# Autodesk Inventor assembly: Assembly1
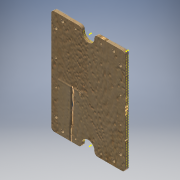
[picture p0: Inventor's stored thumbnail of the model, 180x180]
Saved by Autodesk Inventor 2016 (Build 200138000, 138)
## iProperties
Created: 2022-06-29
Part Number: Assembly1
Document SubType Name: Assembly
Designer: Teemu S.
Author: Teemu S.
## Documents named in this file (4)
- C:\Users\deffener\Documents\Inventor\kajestenciler\Assembly1.iam
- C:\Users\deffener\Documents\Inventor\kajestenciler\base.ipt
- C:\Users\deffener\Documents\Inventor\kajestenciler\side.ipt
- C:\Users\deffener\Documents\Inventor\kajestenciler\pcb-holder.ipt
## Components (5 placed, 3 different names)
1. base:1 — Mate:1, Mate:2, Mate:3
2. side:1 — Mate:5, Mate:6, Mate:7
3. base:2 — Mate:1, Mate:2, Mate:3, Mate:4, Mate:5, Mate:6, Mate:7, Mate:8, Mate:9, Mate:10
4. side:2 — Mate:4, Mate:8, Mate:9
5. pcb-holder:1 — Mate:10
## Relationships (10: Mate 10)
- Mate:1: base:1 ↔ base:2
- Mate:2: base:1 ↔ base:2
- Mate:3: base:1 ↔ base:2
- Mate:4: base:2 ↔ side:2
- Mate:5: side:1 ↔ base:2
- Mate:6: side:1 ↔ base:2
- Mate:7: side:1 ↔ base:2
- Mate:8: base:2 ↔ side:2
- Mate:9: base:2 ↔ side:2
- Mate:10: base:2 ↔ pcb-holder:1
